# Autodesk Inventor assembly: MesaColgada
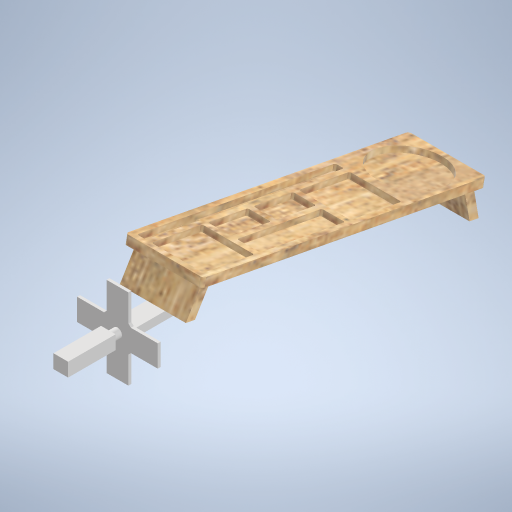
[picture p0: Inventor's stored thumbnail of the model, 512x512]
Saved by Autodesk Inventor 2023 (Build 270158000, 158)
## iProperties
Created: 2023-05-30
Part Number: MesaColgada
Document SubType Name: Assembly
Designer: WIN10
Author: WIN10
## Documents named in this file (3)
- C:\Users\WIN10\DisenoDeProduccion\ModelosCeldaRobotica\MesaColgada.iam
- C:\Users\WIN10\DisenoDeProduccion\ModelosCeldaRobotica\Gancho.ipt
- G:\Unidades compartidas\Amiguitos por siempre\APM 2023-1\Piezas\AssemblyMesa2.iam
## Components (2 placed, 2 different names)
1. Gancho:1 — Coincidencia:1
2. AssemblyMesa2:1 [sub-assembly] — Coincidencia:1
## Relationships (1: Mate 1)
- Coincidencia:1 [Mate]: Gancho:1 ↔ AssemblyMesa2:1
